# Autodesk Inventor assembly: Assembly18
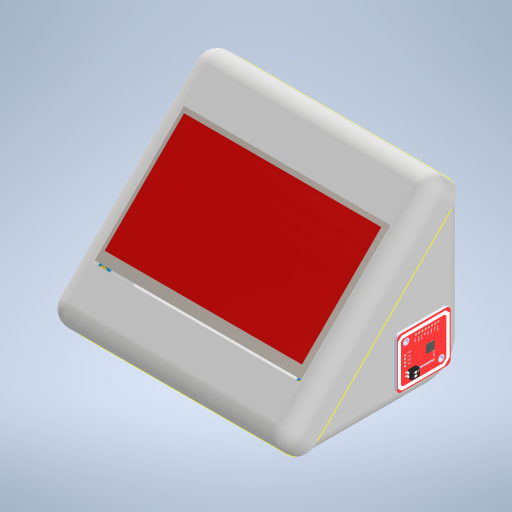
[picture p0: Inventor's stored thumbnail of the model, 512x512]
Saved by Autodesk Inventor 2023 (Build 270158000, 158)
## iProperties
Created: 2023-02-11
Part Number: Assembly18
Document SubType Name: Assembly
Designer: Lauren
Author: Lauren
## Documents named in this file (6)
- C:\Users\Lauren\Documents\due_spring23\ece477\CribCaptain\hardware_assembly\Casing\Assembly18.iam
- C:\Users\Lauren\Documents\due_spring23\ece477\CribCaptain\hardware_assembly\Casing\shell.ipt
- C:\Users\Lauren\Documents\due_spring23\ece477\CribCaptain\hardware_assembly\Casing\outer_casing.ipt
- C:\Users\Lauren\Documents\due_spring23\ece477\CribCaptain\hardware_assembly\keypad-4x4-3.snapshot.1\KlavesniceMembranova.ipt
- C:\Users\Lauren\Documents\due_spring23\ece477\CribCaptain\hardware_assembly\pn532-nfc-rfid-module-v3-kits-1.snapshot.1\PN532_NFC_Assembly.iam
- C:\Users\Lauren\Documents\due_spring23\ece477\CribCaptain\hardware_assembly\7-hdmi-adafruit-touch-screen-1.snapshot.2\HDMI 7po adafruit.ipt
## Components (5 placed, 5 different names)
1. shell:1 — Mate:1, Flush:1, Mate:2, Mate:3, Mate:4, Mate:5, Mate:6, Mate:7, Mate:8
2. outer_casing:1 — Mate:1, Flush:1, Mate:2, Mate:9, Mate:10
3. KlavesniceMembranova:1 — Mate:3, Mate:4, Mate:5
4. PN532_NFC_Assembly:1 [sub-assembly] — Mate:6, Mate:7, Mate:8
5. HDMI 7po adafruit:1 — Mate:9, Mate:10
## Relationships (11: Mate 10, Flush 1)
- Mate:1: shell:1 ↔ outer_casing:1
- Flush:1: shell:1 ↔ outer_casing:1
- Mate:2: shell:1 ↔ outer_casing:1
- Mate:3: shell:1 ↔ KlavesniceMembranova:1
- Mate:4 (6.35 mm): shell:1 ↔ KlavesniceMembranova:1
- Mate:5 (-8.89 mm): shell:1 ↔ KlavesniceMembranova:1
- Mate:6: shell:1 ↔ PN532_NFC_Assembly:1
- Mate:7 (-12.7 mm): shell:1 ↔ PN532_NFC_Assembly:1
- Mate:8 (-12.7 mm): shell:1 ↔ PN532_NFC_Assembly:1
- Mate:9: outer_casing:1 ↔ HDMI 7po adafruit:1
- Mate:10: outer_casing:1 ↔ HDMI 7po adafruit:1
